# Autodesk Inventor assembly: assembly_balancing
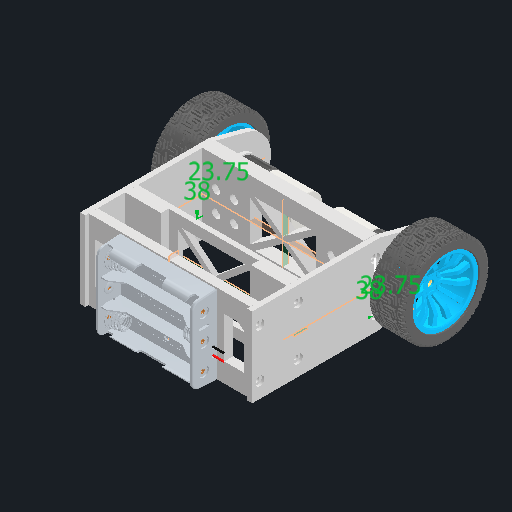
[picture p0: Inventor's stored thumbnail of the model, 512x512]
Saved by Autodesk Inventor 2026 (Build 300175000, 175)
## iProperties
Created: 2026-08-02
Part Number: assembly_balancing
Document SubType Name: Assembly
Designer: imcle
Author: imcle
## Documents named in this file (10)
- D:\Mechatronik\Prj\Self Balancing\self-balancing-robot\hardware\assembly_balancing.iam
- D:\Mechatronik\Prj\Self Balancing\self-balancing-robot\hardware\Library\motor\25ga-370-280-rpm-dc Motor.ipt
- D:\Mechatronik\Prj\Self Balancing\self-balancing-robot\hardware\Library\do_ga'\do_ga.ipt
- D:\Mechatronik\Prj\Self Balancing\self-balancing-robot\hardware\parts\plate.ipt
- D:\Mechatronik\Prj\Self Balancing\self-balancing-robot\hardware\Library\wheel\65mm蓝色轮胎总装-实际外径68mm.ipt
- D:\Mechatronik\Prj\Self Balancing\mpu6050\MPU6050\MPU6050\MPU6050.ipt
- D:\Mechatronik\Prj\Self Balancing\self-balancing-robot\hardware\parts\plate_base.ipt
- D:\Mechatronik\Prj\Self Balancing\self-balancing-robot\hardware\Library\battery_case\batteryCase18650x3.ipt
- D:\Mechatronik\Prj\Self Balancing\self-balancing-robot\hardware\parts\base2.ipt
- D:\Mechatronik\Prj\Self Balancing\self-balancing-robot\hardware\parts\base3.ipt
## Components (13 placed, 9 different names)
1. 25ga-370-280-rpm-dc Motor:1 — Rigid:1, Rotational:1
2. 25ga-370-280-rpm-dc Motor:2 — Rigid:2, Rotational:2
3. do_ga:1 — Rigid:1, Rigid:3, Rigid:5
4. do_ga:2 — Rigid:2, Rigid:4, Rigid:6
5. plate:2 — Rigid:3, Rigid:4
6. 65mm蓝色轮胎总装-实际外径68mm:1 — Rotational:1
7. 65mm蓝色轮胎总装-实际外径68mm:2 — Rotational:2
8. MPU6050:1
9. plate_base:1 — Rigid:5
10. plate_base:2 — Rigid:6, Rigid:7, Rigid:8
11. batteryCase18650x3:1 — Rigid:9
12. base2:1 — Rigid:7
13. base3:1 — Rigid:8, Rigid:9
## Relationships (11: WeldJoint 9, RevoluteJoint 2)
- Rigid:1 [WeldJoint]: 25ga-370-280-rpm-dc Motor:1 ↔ do_ga:1
- Rigid:2 [WeldJoint]: 25ga-370-280-rpm-dc Motor:2 ↔ do_ga:2
- Rigid:3 [WeldJoint]: do_ga:1 ↔ plate:2
- Rigid:4 [WeldJoint]: do_ga:2 ↔ plate:2
- Rotational:1 [RevoluteJoint]: 25ga-370-280-rpm-dc Motor:1 ↔ 65mm蓝色轮胎总装-实际外径68mm:1
- Rigid:5 [WeldJoint]: do_ga:1 ↔ plate_base:1
- Rigid:6 [WeldJoint]: do_ga:2 ↔ plate_base:2
- Rotational:2 [RevoluteJoint]: 25ga-370-280-rpm-dc Motor:2 ↔ 65mm蓝色轮胎总装-实际外径68mm:2
- Rigid:7 [WeldJoint]: plate_base:2 ↔ base2:1
- Rigid:8 [WeldJoint]: plate_base:2 ↔ base3:1
- Rigid:9 [WeldJoint]: batteryCase18650x3:1 ↔ base3:1
